# Autodesk Inventor assembly: intake_MIR
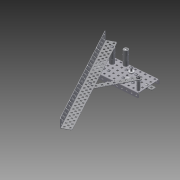
[picture p0: Inventor's stored thumbnail of the model, 180x180]
Saved by Autodesk Inventor 2014 (Build 180170000, 170)
## iProperties
Created: 2013-09-20
Part Number: intake_MIR
Document SubType Name: Assembly
Designer: Ryan
Author: Ryan
## Documents named in this file (18)
- C:\Users\Ryan\Desktop\sw\toss up robot intake\intake_MIR.iam
- C:\Users\Ryan\Desktop\sw\lib\Aperture VEX CAD Library\Metal\C Channel\5 x 10.ipt
- C:\Users\Ryan\Desktop\sw\lib\Aperture VEX CAD Library\Bearing Blocks\Bearing Block.ipt
- C:\Users\Ryan\Desktop\sw\lib\Aperture VEX CAD Library\Hardware\8-32\locknut (copy).ipt
- C:\Users\Ryan\Desktop\sw\lib\Aperture VEX CAD Library\Hardware\8-32\8-32_.500.ipt
- C:\Users\Ryan\Desktop\sw\lib\Aperture VEX CAD Library\Spacers\SPACER-0500-0500.ipt
- C:\Users\Ryan\Desktop\sw\lib\Aperture VEX CAD Library\Hardware\8-32\8-32_1.750.ipt
- C:\Users\Ryan\Desktop\sw\lib\Aperture VEX CAD Library\Hardware\8-32\8-32_2.000.ipt
- C:\Users\Ryan\Desktop\sw\lib\custom parts\1x2 bar.ipt
- C:\Users\Ryan\Desktop\sw\lib\Aperture VEX CAD Library\Hardware\8-32\8-32_.375.ipt
- C:\Users\Ryan\Desktop\sw\lib\Aperture VEX CAD Library\Metal\L Bar\2 x 25.ipt
- C:\Users\Ryan\Desktop\sw\lib\Aperture VEX CAD Library\Standoffs\BEAM-1000.ipt
- C:\Users\Ryan\Desktop\sw\lib\Aperture VEX CAD Library\Spacers\SPACER-0500-0125.ipt
- C:\Users\Ryan\Desktop\sw\lib\Aperture VEX CAD Library\Hardware\8-32\8-32_1.500.ipt
- C:\Users\Ryan\Desktop\sw\lib\custom parts\1x9.ipt
- C:\Users\Ryan\Desktop\sw\lib\Aperture VEX CAD Library\Spacers\SPACER-0500-0250.ipt
- C:\Users\Ryan\Desktop\sw\lib\Aperture VEX CAD Library\Hardware\8-32\locknut (copy)_MIR.ipt
- C:\Users\Ryan\Desktop\sw\lib\Aperture VEX CAD Library\Hardware\8-32\8-32_.875.ipt
## Components (45 placed, 17 different names)
1. 5 x 10:1 — Mate:1, Mate:24, Mate:27, Mate:9, Mate:5, Mate:19, Mate:26, Mate:25, Mate:23, Mate:22, Mate:21, Mate:20, Mate:12, Mate:11, Mate:10, Mate:8, Mate:7, Mate:4, Mate:3, Mate:36, Mate:30, Mate:32, Mate:33, Mate:39, Mate:40, Mate:46, Flush:58, Flush:57, Mate:55, Mate:56, Mate:67, Mate:66, Mate:65, Mate:71, Mate:86, Mate:88, Mate:90
2. Bearing Block:1 — Mate:1, Mate:37, Mate:14, Mate:13, Mate:20, Mate:4, Mate:3, Mate:38, Mate:91
3. locknut (copy):1 — Mate:24, Mate:26, Mate:25, Mate:41
4. 8-32_.500:1 — Mate:37, Mate:27
5. Bearing Block:2 — Mate:9, Mate:16, Mate:15, Mate:12, Mate:11, Mate:10, Mate:29, Mate:31, Mate:89
6. Bearing Block:3 — Mate:5, Mate:18, Mate:17, Mate:21, Mate:8, Mate:7, Mate:35, Mate:34, Mate:87
7. locknut (copy):2 — Mate:19, Mate:23, Mate:22, Mate:47
8. 8-32_.500:2 — Mate:36, Mate:35
9. 8-32_.500:3 — Mate:30, Mate:29
10. 8-32_.500:4 — Mate:32, Mate:31
11. 8-32_.500:5 — Mate:34, Mate:33
12. 8-32_.500:6 — Mate:39, Mate:38
13. SPACER-0500-0500:1 — Mate:51, Mate:50, Mate:53, Mate:52
14. SPACER-0500-0500:2 — Mate:41, Mate:40, Mate:43, Mate:42, Mate:45
15. SPACER-0500-0500:3 — Mate:43, Mate:42, Mate:44
16. SPACER-0500-0500:4 — Mate:51, Mate:50, Mate:49, Mate:48
17. SPACER-0500-0500:5 — Mate:49, Mate:48, Mate:47, Mate:46
18. SPACER-0500-0500:6 — Mate:45, Mate:44, Mate:54, Mate:61
19. 8-32_1.750:1 — Mate:53, Mate:52
20. 8-32_2.000:1 — Mate:54, Mate:64, Mate:63, Mate:62
21. 1x2 bar:1 — Flush:58, Flush:57, Mate:55, Mate:58, Mate:57, Mate:59
22. 8-32_.375:1 — Mate:58, Mate:57, Mate:56, Mate:60
23. locknut (copy):6 — Mate:60, Mate:59
24. 2 x 25:1 — Mate:64, Mate:63, Mate:62, Mate:61, Mate:79, Mate:78, Mate:77, Mate:82
25. BEAM-1000:1 — Mate:67, Mate:66, Mate:65, Mate:69, Mate:68
26. SPACER-0500-0125:1 — Mate:69, Mate:68, Mate:70, Mate:74
27. 8-32_1.500:1 — Mate:71, Mate:70, Mate:73, Mate:72, Mate:76
28. 1x9:1 — Mate:74, Mate:73, Mate:72, Mate:75, Mate:81, Mate:80, Mate:85
29. locknut (copy):7 — Mate:76, Mate:75
30. SPACER-0500-0250:1 — Mate:81, Mate:80, Mate:79, Mate:78, Mate:77, Mate:83
31. 8-32_.500:7 — Mate:83, Mate:82, Mate:84
32. locknut (copy)_MIR:1 — Mate:85, Mate:84
33. SPACER-0500-0125:2 — Mate:87, Mate:86
34. SPACER-0500-0125:3 — Mate:89, Mate:88, Mate:93, Mate:92
35. SPACER-0500-0125:4 — Mate:91, Mate:90
36. 8-32_.875:1 — Mate:93, Mate:92
37. locknut (copy):4 — Mate:14, Mate:13
38. locknut (copy):8
39. locknut (copy):9
40. locknut (copy):3 — Mate:16, Mate:15
41. locknut (copy):10
42. locknut (copy):11
43. locknut (copy):5 — Mate:18, Mate:17
44. locknut (copy):12
45. locknut (copy):13
## Component patterns: (3 elements, first: locknut (copy):4), (3 elements, first: locknut (copy):3), (3 elements, first: locknut (copy):5)
## Relationships (92: Mate 90, Flush 2)
- Mate:1: 5 x 10:1 ↔ Bearing Block:1
- Mate:24: 5 x 10:1 ↔ locknut (copy):1
- Mate:37: Bearing Block:1 ↔ 8-32_.500:1
- Mate:27: 5 x 10:1 ↔ 8-32_.500:1
- Mate:9: 5 x 10:1 ↔ Bearing Block:2
- Mate:5: 5 x 10:1 ↔ Bearing Block:3
- Mate:19: 5 x 10:1 ↔ locknut (copy):2
- Mate:16: Bearing Block:2 ↔ locknut (copy):3
- Mate:15: Bearing Block:2 ↔ locknut (copy):3
- Mate:14: Bearing Block:1 ↔ locknut (copy):4
- Mate:13: Bearing Block:1 ↔ locknut (copy):4
- Mate:18: Bearing Block:3 ↔ locknut (copy):5
- Mate:17: Bearing Block:3 ↔ locknut (copy):5
- Mate:26 (2.3114 mm): 5 x 10:1 ↔ locknut (copy):1
- Mate:25 (2.3114 mm): 5 x 10:1 ↔ locknut (copy):1
- Mate:23 (2.3114 mm): 5 x 10:1 ↔ locknut (copy):2
- Mate:22 (2.3114 mm): 5 x 10:1 ↔ locknut (copy):2
- Mate:21 (2.3114 mm): 5 x 10:1 ↔ Bearing Block:3
- Mate:20 (2.3114 mm): 5 x 10:1 ↔ Bearing Block:1
- Mate:12 (2.3114 mm): 5 x 10:1 ↔ Bearing Block:2
- Mate:11 (2.3114 mm): 5 x 10:1 ↔ Bearing Block:2
- Mate:10 (2.3114 mm): 5 x 10:1 ↔ Bearing Block:2
- Mate:8 (2.3114 mm): 5 x 10:1 ↔ Bearing Block:3
- Mate:7 (2.3114 mm): 5 x 10:1 ↔ Bearing Block:3
- Mate:4 (2.3114 mm): 5 x 10:1 ↔ Bearing Block:1
- Mate:3 (2.3114 mm): 5 x 10:1 ↔ Bearing Block:1
- Mate:36: 5 x 10:1 ↔ 8-32_.500:2
- Mate:35: Bearing Block:3 ↔ 8-32_.500:2
- Mate:30: 5 x 10:1 ↔ 8-32_.500:3
- Mate:29: Bearing Block:2 ↔ 8-32_.500:3
- Mate:32: 5 x 10:1 ↔ 8-32_.500:4
- Mate:31: Bearing Block:2 ↔ 8-32_.500:4
- Mate:34: Bearing Block:3 ↔ 8-32_.500:5
- Mate:33: 5 x 10:1 ↔ 8-32_.500:5
- Mate:39: 5 x 10:1 ↔ 8-32_.500:6
- Mate:38: Bearing Block:1 ↔ 8-32_.500:6
- Mate:41: locknut (copy):1 ↔ SPACER-0500-0500:2
- Mate:40: 5 x 10:1 ↔ SPACER-0500-0500:2
- Mate:43: SPACER-0500-0500:2 ↔ SPACER-0500-0500:3
- Mate:42: SPACER-0500-0500:2 ↔ SPACER-0500-0500:3
- Mate:51: SPACER-0500-0500:1 ↔ SPACER-0500-0500:4
- Mate:50: SPACER-0500-0500:1 ↔ SPACER-0500-0500:4
- Mate:49: SPACER-0500-0500:4 ↔ SPACER-0500-0500:5
- Mate:48: SPACER-0500-0500:4 ↔ SPACER-0500-0500:5
- Mate:47: locknut (copy):2 ↔ SPACER-0500-0500:5
- Mate:46: 5 x 10:1 ↔ SPACER-0500-0500:5
- Mate:45: SPACER-0500-0500:2 ↔ SPACER-0500-0500:6
- Mate:44: SPACER-0500-0500:3 ↔ SPACER-0500-0500:6
- Mate:53: SPACER-0500-0500:1 ↔ 8-32_1.750:1
- Mate:52: SPACER-0500-0500:1 ↔ 8-32_1.750:1
- Mate:54: SPACER-0500-0500:6 ↔ 8-32_2.000:1
- Flush:58: 5 x 10:1 ↔ 1x2 bar:1
- Flush:57: 5 x 10:1 ↔ 1x2 bar:1
- Mate:55: 5 x 10:1 ↔ 1x2 bar:1
- Mate:58 (2.3114 mm): 1x2 bar:1 ↔ 8-32_.375:1
- Mate:57 (2.3114 mm): 1x2 bar:1 ↔ 8-32_.375:1
- Mate:56: 5 x 10:1 ↔ 8-32_.375:1
- Mate:60: 8-32_.375:1 ↔ locknut (copy):6
- Mate:59: 1x2 bar:1 ↔ locknut (copy):6
- Mate:64: 8-32_2.000:1 ↔ 2 x 25:1
- Mate:63 (2.3114 mm): 8-32_2.000:1 ↔ 2 x 25:1
- Mate:62 (2.3114 mm): 8-32_2.000:1 ↔ 2 x 25:1
- Mate:61: SPACER-0500-0500:6 ↔ 2 x 25:1
- Mate:67 (2.3114 mm): 5 x 10:1 ↔ BEAM-1000:1
- Mate:66 (2.3114 mm): 5 x 10:1 ↔ BEAM-1000:1
- Mate:65: 5 x 10:1 ↔ BEAM-1000:1
- Mate:69: BEAM-1000:1 ↔ SPACER-0500-0125:1
- Mate:68: BEAM-1000:1 ↔ SPACER-0500-0125:1
- Mate:71: 5 x 10:1 ↔ 8-32_1.500:1
- Mate:70: SPACER-0500-0125:1 ↔ 8-32_1.500:1
- Mate:74: SPACER-0500-0125:1 ↔ 1x9:1
- Mate:73 (2.3114 mm): 8-32_1.500:1 ↔ 1x9:1
- Mate:72 (2.3114 mm): 8-32_1.500:1 ↔ 1x9:1
- Mate:76: 8-32_1.500:1 ↔ locknut (copy):7
- Mate:75: 1x9:1 ↔ locknut (copy):7
- Mate:81 (2.3114 mm): 1x9:1 ↔ SPACER-0500-0250:1
- Mate:80 (2.3114 mm): 1x9:1 ↔ SPACER-0500-0250:1
- Mate:79 (2.3114 mm): 2 x 25:1 ↔ SPACER-0500-0250:1
- Mate:78 (2.3114 mm): 2 x 25:1 ↔ SPACER-0500-0250:1
- Mate:77: 2 x 25:1 ↔ SPACER-0500-0250:1
- Mate:83: SPACER-0500-0250:1 ↔ 8-32_.500:7
- Mate:82: 2 x 25:1 ↔ 8-32_.500:7
- Mate:85: 1x9:1 ↔ locknut (copy)_MIR:1
- Mate:84: 8-32_.500:7 ↔ locknut (copy)_MIR:1
- Mate:87: Bearing Block:3 ↔ SPACER-0500-0125:2
- Mate:86: 5 x 10:1 ↔ SPACER-0500-0125:2
- Mate:89: Bearing Block:2 ↔ SPACER-0500-0125:3
- Mate:88: 5 x 10:1 ↔ SPACER-0500-0125:3
- Mate:91: Bearing Block:1 ↔ SPACER-0500-0125:4
- Mate:90: 5 x 10:1 ↔ SPACER-0500-0125:4
- Mate:93 (7.9375 mm): SPACER-0500-0125:3 ↔ 8-32_.875:1
- Mate:92: SPACER-0500-0125:3 ↔ 8-32_.875:1
